# Autodesk Inventor assembly: assembly_v2
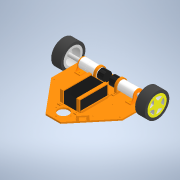
[picture p0: Inventor's stored thumbnail of the model, 180x180]
Saved by Autodesk Inventor 2020.3 (Build 243373000, 373)
## iProperties
Created: 2020-06-30
Part Number: assembly_v2
Document SubType Name: Assembly
Designer: Devin
Author: Devin
## Documents named in this file (8)
- C:\Github\robo_car\mechanical\assembly_v2.iam
- C:\Github\robo_car\mechanical\bp_v3.ipt
- C:\Github\robo_car\mechanical\main_motor_mount.ipt
- C:\Github\robo_car\mechanical\gearmotor.ipt
- C:\Github\robo_car\mechanical\motor_support_v2.ipt
- C:\Github\robo_car\mechanical\tenergy_nimh_2200.ipt
- C:\Github\robo_car\mechanical\battery_pack_clamp_v2.ipt
- C:\Github\robo_car\mechanical\mock_wheel.ipt
## Components (12 placed, 7 different names)
1. bp_v3:1 — Mate:1, Mate:2, Mate:3, Mate:4, Mate:5, Mate:6, Mate:10, Mate:11, Flush:1, Flush:2, Mate:12, Mate:13, Mate:15, Mate:16, Flush:3, Flush:4, Mate:18, Mate:20, Mate:21, Mate:22, Flush:24
2. main_motor_mount:1 — Mate:1, Mate:2, Mate:3, Mate:8, Cylindrical:1
3. main_motor_mount:2 — Mate:4, Mate:5, Mate:6, Mate:9, Cylindrical:2
4. gearmotor:1 — Mate:9, Cylindrical:2, Cylindrical:4, Mate:24
5. gearmotor:2 — Mate:8, Cylindrical:1, Cylindrical:3, Mate:23
6. motor_support_v2:1 — Flush:2, Mate:12, Mate:13
7. motor_support_v2:2 — Mate:10, Mate:11, Flush:1
8. tenergy_nimh_2200:1 — Mate:15, Mate:16, Flush:3, Mate:17, Mate:19
9. battery_pack_clamp_v2:1 — Mate:19, Mate:20, Mate:21
10. battery_pack_clamp_v2:2 — Mate:17, Flush:4, Mate:18
11. mock_wheel:1 — Cylindrical:4, Mate:24
12. mock_wheel:2 — Cylindrical:3, Mate:23
## Relationships (31: Mate 22, Flush 5, CylindricalJoint 4)
- Mate:1: bp_v3:1 ↔ main_motor_mount:1
- Mate:2: bp_v3:1 ↔ main_motor_mount:1
- Mate:3: bp_v3:1 ↔ main_motor_mount:1
- Mate:4: bp_v3:1 ↔ main_motor_mount:2
- Mate:5: bp_v3:1 ↔ main_motor_mount:2
- Mate:6: bp_v3:1 ↔ main_motor_mount:2
- Mate:8: main_motor_mount:1 ↔ gearmotor:2
- Cylindrical:1: main_motor_mount:1 ↔ gearmotor:2
- Mate:9: main_motor_mount:2 ↔ gearmotor:1
- Cylindrical:2: main_motor_mount:2 ↔ gearmotor:1
- Mate:10: bp_v3:1 ↔ motor_support_v2:2
- Mate:11: bp_v3:1 ↔ motor_support_v2:2
- Flush:1: bp_v3:1 ↔ motor_support_v2:2
- Flush:2: bp_v3:1 ↔ motor_support_v2:1
- Mate:12: bp_v3:1 ↔ motor_support_v2:1
- Mate:13: bp_v3:1 ↔ motor_support_v2:1
- Mate:15: bp_v3:1 ↔ tenergy_nimh_2200:1
- Mate:16: bp_v3:1 ↔ tenergy_nimh_2200:1
- Flush:3: bp_v3:1 ↔ tenergy_nimh_2200:1
- Mate:17: tenergy_nimh_2200:1 ↔ battery_pack_clamp_v2:2
- Flush:4 (2.4 mm): bp_v3:1 ↔ battery_pack_clamp_v2:2
- Mate:18: bp_v3:1 ↔ battery_pack_clamp_v2:2
- Mate:19: tenergy_nimh_2200:1 ↔ battery_pack_clamp_v2:1
- Mate:20: bp_v3:1 ↔ battery_pack_clamp_v2:1
- Mate:21: bp_v3:1 ↔ battery_pack_clamp_v2:1
- Mate:22: bp_v3:1
- Flush:24: bp_v3:1
- Cylindrical:3: gearmotor:2 ↔ mock_wheel:2
- Mate:23: gearmotor:2 ↔ mock_wheel:2
- Cylindrical:4: gearmotor:1 ↔ mock_wheel:1
- Mate:24: gearmotor:1 ↔ mock_wheel:1
